# Autodesk Inventor assembly: FULL SWERVE DRIVE ASSEMBLY!  4!
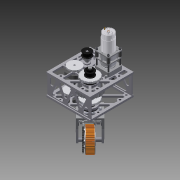
[picture p0: Inventor's stored thumbnail of the model, 180x180]
Saved by Autodesk Inventor 2012 (Build 160160000, 160)
## iProperties
Created: 2013-01-01
Part Number: FULL SWERVE DRIVE ASSEMBLY!  4!
Document SubType Name: Assembly
Designer: Bryce
Author: Bryce
## Documents named in this file (16)
- C:\Users\Bryce\Dropbox\Inventor Design Project Files\Independent Swerves\Inventor 2012\FULL SWERVE DRIVE ASSEMBLY!  4!.iam
- C:\Users\Bryce\Dropbox\Inventor Design Project Files\Independent Swerves\Inventor 2012\collar bearing systom.ipt
- C:\Users\Bryce\Dropbox\Inventor Design Project Files\Independent Swerves\Imported Components\CIM Motor.iam
- C:\Users\Bryce\Dropbox\Inventor Design Project Files\Independent Swerves\Inventor 2012\turn encoder assembly.iam
- C:\Users\Bryce\Dropbox\Inventor Design Project Files\Independent Swerves\Imported Components\Imported Components\48-5m09-6a5\48-5m09-6a5.ipt
- C:\Users\Bryce\Dropbox\Inventor Design Project Files\Independent Swerves\Inventor 2012\frame assembly 2.iam
- C:\Users\Bryce\Dropbox\Inventor Design Project Files\Independent Swerves\Imported Components\encoder gear drive.ipt
- C:\Users\Bryce\Dropbox\Inventor Design Project Files\Independent Swerves\Imported Components\encoder gear turn.ipt
- C:\Users\Bryce\Dropbox\Inventor Design Project Files\Independent Swerves\Imported Components\15T plastick sprocket .375.ipt
- C:\Users\Bryce\Dropbox\Inventor Design Project Files\Independent Swerves\Imported Components\15T plastick sprocket 8mm.ipt
- C:\Users\Bryce\Dropbox\Inventor Design Project Files\Independent Swerves\Imported Components\15T plastick sprocket .375 threaded.ipt
- C:\Users\Bryce\Dropbox\Inventor Design Project Files\Independent Swerves\Inventor 2012\sprocket hub adaptor.ipt
- C:\Users\Bryce\Dropbox\Inventor Design Project Files\Independent Swerves\Inventor 2012\tensioning wedge.ipt
- C:\Users\Bryce\Dropbox\Inventor Design Project Files\Independent Swerves\Imported Components\BD Gearbox and Bracket Assy 4.iam
- C:\Users\Bryce\Dropbox\Inventor Design Project Files\Independent Swerves\Inventor 2012\Lower box main assembly 4.iam
- C:\Users\Bryce\Dropbox\Inventor Design Project Files\Independent Swerves\Inventor 2012\upper gearbox frame 3.ipt
## Components (18 placed, 15 different names)
1. upper gearbox frame 3:1 — Mate:1, Mate:2, Mate:3, Mate:4, Mate:11, Mate:15, Mate:16, Mate:17, Mate:18, Angle:2, Mate:24, Mate:25, Mate:26, Mate:40, Mate:41, Flush:15, Flush:16, Mate:50, Mate:51, Mate:52, Mate:53, Mate:54, Mate:55, Mate:56, Mate:58
2. collar bearing systom:1 — Mate:1, Mate:2, Flush:1
3. collar bearing systom:2 — Mate:3, Mate:4, Mate:5
4. Lower box main assembly 4:1 [sub-assembly] — Mate:5, Flush:1, Mate:23, Flush:4, Mate:36, Flush:10, Mate:37, Mate:43, Flush:12
5. BD Gearbox and Bracket Assy 4:1 [sub-assembly] — Mate:40, Mate:41, Mate:46, Mate:47, Mate:54, Mate:58
6. CIM Motor:1 [sub-assembly] — Mate:11, Mate:42, Mate:55, Mate:56
7. turn encoder assembly:1 [sub-assembly] — Mate:17, Mate:18, Angle:1, Angle:2, Rotation:3, Rotation:4
8. turn encoder assembly:2 [sub-assembly] — Mate:15, Mate:16, Angle:1, Rotation:2
9. encoder gear turn:1 — Mate:36, Flush:10, Rotation:3, Rotation:4
10. 48-5m09-6a5:1 — Mate:23, Flush:4, Flush:17
11. frame assembly 2:1 [sub-assembly] — Mate:24, Mate:25, Mate:26
12. 15T plastick sprocket .375 threaded:1 — Mate:46, Mate:47, Flush:17
13. 15T plastick sprocket 8mm:1 — Mate:42, Mate:48, Mate:49, Flush:13, Flush:14, Rotation:7, Mate:57
14. encoder gear drive:1 — Mate:37, Rotation:2, Mate:44, Rotation:6
15. 15T plastick sprocket .375:1 — Mate:43, Flush:12, Mate:44, Rotation:6, Flush:14, Rotation:7, Mate:57
16. sprocket hub adaptor:1 — Mate:48, Mate:49, Flush:13
17. tensioning wedge:1 — Flush:15, Mate:50, Mate:52
18. tensioning wedge:2 — Flush:16, Mate:51, Mate:53
## Relationships (53: Mate 34, Flush 11, RelateRotation 6, Angle 2)
- Mate:1: upper gearbox frame 3:1 ↔ collar bearing systom:1
- Mate:2: upper gearbox frame 3:1 ↔ collar bearing systom:1
- Mate:3: upper gearbox frame 3:1 ↔ collar bearing systom:2
- Mate:4: upper gearbox frame 3:1 ↔ collar bearing systom:2
- Mate:5: collar bearing systom:2 ↔ Lower box main assembly 4:1
- Flush:1 (-1.27 mm): collar bearing systom:1 ↔ Lower box main assembly 4:1
- Mate:11: upper gearbox frame 3:1 ↔ CIM Motor:1
- Mate:15: upper gearbox frame 3:1 ↔ turn encoder assembly:2
- Mate:16: upper gearbox frame 3:1 ↔ turn encoder assembly:2
- Mate:17: upper gearbox frame 3:1 ↔ turn encoder assembly:1
- Mate:18: upper gearbox frame 3:1 ↔ turn encoder assembly:1
- [Flush]: turn encoder assembly:1 ↔ encoder gear turn:1
- Mate:23: Lower box main assembly 4:1 ↔ 48-5m09-6a5:1
- Flush:4: Lower box main assembly 4:1 ↔ 48-5m09-6a5:1
- Angle:1 (0 deg): turn encoder assembly:1 ↔ turn encoder assembly:2
- Angle:2 (0 deg): upper gearbox frame 3:1 ↔ turn encoder assembly:1
- Mate:24: upper gearbox frame 3:1 ↔ frame assembly 2:1
- Mate:25: upper gearbox frame 3:1 ↔ frame assembly 2:1
- Mate:26: upper gearbox frame 3:1 ↔ frame assembly 2:1
- [Flush]: turn encoder assembly:2 ↔ encoder gear drive:1
- Mate:36: Lower box main assembly 4:1 ↔ encoder gear turn:1
- Flush:10: Lower box main assembly 4:1 ↔ encoder gear turn:1
- Mate:37: Lower box main assembly 4:1 ↔ encoder gear drive:1
- Rotation:2 [RelateRotation] (1 ul): turn encoder assembly:2 ↔ encoder gear drive:1
- Rotation:3 [RelateRotation] (1 ul): turn encoder assembly:1 ↔ encoder gear turn:1
- Rotation:4 [RelateRotation] (1 ul): turn encoder assembly:1 ↔ encoder gear turn:1
- Mate:40 (3.175 mm): upper gearbox frame 3:1 ↔ BD Gearbox and Bracket Assy 4:1
- Mate:41 (3.175 mm): upper gearbox frame 3:1 ↔ BD Gearbox and Bracket Assy 4:1
- [RelateRotation] (0.3333 ul): 48-5m09-6a5:1 ↔ 15T plastick sprocket .375 threaded:1
- Mate:42: CIM Motor:1 ↔ 15T plastick sprocket 8mm:1
- Mate:43: Lower box main assembly 4:1 ↔ 15T plastick sprocket .375:1
- Flush:12: Lower box main assembly 4:1 ↔ 15T plastick sprocket .375:1
- Mate:44: encoder gear drive:1 ↔ 15T plastick sprocket .375:1
- Rotation:6 [RelateRotation] (1 ul): encoder gear drive:1 ↔ 15T plastick sprocket .375:1
- Mate:46: BD Gearbox and Bracket Assy 4:1 ↔ 15T plastick sprocket .375 threaded:1
- Mate:47: BD Gearbox and Bracket Assy 4:1 ↔ 15T plastick sprocket .375 threaded:1
- Mate:48: 15T plastick sprocket 8mm:1 ↔ sprocket hub adaptor:1
- Mate:49: 15T plastick sprocket 8mm:1 ↔ sprocket hub adaptor:1
- Flush:13: 15T plastick sprocket 8mm:1 ↔ sprocket hub adaptor:1
- Flush:14: 15T plastick sprocket 8mm:1 ↔ 15T plastick sprocket .375:1
- Flush:15 (-6.35 mm): upper gearbox frame 3:1 ↔ tensioning wedge:1
- Flush:16 (-6.35 mm): upper gearbox frame 3:1 ↔ tensioning wedge:2
- Mate:50: upper gearbox frame 3:1 ↔ tensioning wedge:1
- Mate:51: upper gearbox frame 3:1 ↔ tensioning wedge:2
- Mate:52: upper gearbox frame 3:1 ↔ tensioning wedge:1
- Mate:53: upper gearbox frame 3:1 ↔ tensioning wedge:2
- Flush:17 (0.254 mm): 48-5m09-6a5:1 ↔ 15T plastick sprocket .375 threaded:1
- Mate:54: upper gearbox frame 3:1 ↔ BD Gearbox and Bracket Assy 4:1
- Rotation:7 [RelateRotation] (1 ul): 15T plastick sprocket 8mm:1 ↔ 15T plastick sprocket .375:1
- Mate:55 (2.54 mm): upper gearbox frame 3:1 ↔ CIM Motor:1
- Mate:56 (2.54 mm): upper gearbox frame 3:1 ↔ CIM Motor:1
- Mate:57 (84.201 mm): 15T plastick sprocket 8mm:1 ↔ 15T plastick sprocket .375:1
- Mate:58 (9.525 mm): upper gearbox frame 3:1 ↔ BD Gearbox and Bracket Assy 4:1
